# Autodesk Inventor assembly: Body
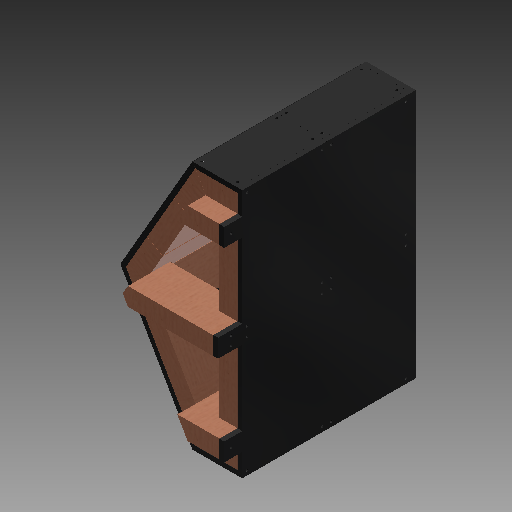
[picture p0: Inventor's stored thumbnail of the model, 512x512]
Saved by Autodesk Inventor 2017 (Build 210142000, 142)
## iProperties
Created: 2018-10-18
Part Number: Body
Document SubType Name: Assembly
Designer: Dell
Author: Dell
## Documents named in this file (3)
- C:\Users\Dell\Documents\GitHub\tr2\Body\Body.iam
- C:\Users\Dell\Documents\GitHub\tr2\Body\Body Cover Assembly.iam
- C:\Users\Dell\Documents\GitHub\tr2\Body\Body Chassis Assembly.iam
## Components (2 placed, 2 different names)
1. Body Cover Assembly:1 [sub-assembly]
2. Body Chassis Assembly:1 [sub-assembly]
## Relationships (15: Mate 15)
- [Mate]: Body Cover Assembly:1 ↔ Body Chassis Assembly:1
- [Mate]: Body Cover Assembly:1 ↔ Body Chassis Assembly:1
- [Mate]: Body Cover Assembly:1 ↔ Body Chassis Assembly:1
- [Mate]: Body Cover Assembly:1 ↔ Body Chassis Assembly:1
- [Mate]: Body Cover Assembly:1 ↔ Body Chassis Assembly:1
- [Mate]: Body Cover Assembly:1 ↔ Body Chassis Assembly:1
- [Mate]: Body Cover Assembly:1 ↔ Body Chassis Assembly:1
- [Mate]: Body Cover Assembly:1 ↔ Body Chassis Assembly:1
- [Mate]: Body Cover Assembly:1 ↔ Body Chassis Assembly:1
- [Mate]: Body Cover Assembly:1 ↔ Body Chassis Assembly:1
- [Mate]: Body Cover Assembly:1 ↔ Body Chassis Assembly:1
- [Mate]: Body Cover Assembly:1 ↔ Body Chassis Assembly:1
- [Mate]: Body Cover Assembly:1 ↔ Body Chassis Assembly:1
- [Mate]: Body Cover Assembly:1 ↔ Body Chassis Assembly:1
- [Mate]: Body Cover Assembly:1 ↔ Body Chassis Assembly:1
